# Autodesk Inventor assembly: BobbinGuide
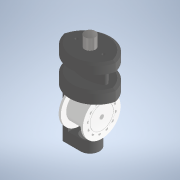
[picture p0: Inventor's stored thumbnail of the model, 180x180]
Saved by Autodesk Inventor 2022 (Build 260153070, 153G)
## iProperties
Created: 2020-03-09
Part Number: BobbinGuide
Document SubType Name: Assembly
Designer: elmar
Author: elmar
## Documents named in this file (6)
- D:\FourWireBraidingMachine\MetalCableBraider\Carriage.iam
- D:\FourWireBraidingMachine\MetalCableBraider\SpoolHolder.ipt
- D:\FourWireBraidingMachine\MetalCableBraider\Spool.ipt
- D:\FourWireBraidingMachine\MetalCableBraider\Spring.ipt
- D:\FourWireBraidingMachine\MetalCableBraider\SpoolSpringBushing.ipt
- D:\FourWireBraidingMachine\MetalCableBraider\M8_34mmRod.ipt
## Components (5 placed, 5 different names)
1. SpoolHolder:1 — Insert:20, Insert:23
2. Spool:1 — Mate:1, Mate:5, Insert:20, Insert:22
3. Spring:1 — Mate:1, Mate:5
4. SpoolSpringBushing:1 — Insert:22
5. M8_34mmRod:1 — Insert:23
## Relationships (5: Insert 3, Mate 2)
- Mate:1: Spool:1 ↔ Spring:1
- Mate:5: Spool:1 ↔ Spring:1
- Insert:20: SpoolHolder:1 ↔ Spool:1
- Insert:22: Spool:1 ↔ SpoolSpringBushing:1
- Insert:23: SpoolHolder:1 ↔ M8_34mmRod:1
